# Autodesk Inventor assembly: assembly
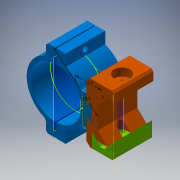
[picture p0: Inventor's stored thumbnail of the model, 180x180]
Saved by Autodesk Inventor 2019 (Build 230136000, 136)
## iProperties
Created: 2021-10-21
Part Number: assembly
Material: Genérico
Document SubType Name: Assembly
Designer: Juan M. Casillas
Author: Juan M. Casillas
## Documents named in this file (4)
- K:\3DPrinting\3DModels\RIS\assembly.iam
- K:\3DPrinting\3DModels\RIS\bolt_part.ipt
- K:\3DPrinting\3DModels\RIS\nut_part.ipt
- K:\3DPrinting\3DModels\RIS\flashlight_support.ipt
## Components (3 placed, 3 different names)
1. bolt_part:1 — Rigid:1, Rigid:2
2. nut_part:1 — Rigid:1
3. flashlight_support:1 — Rigid:2
## Relationships (2: WeldJoint 2)
- Rigid:1 [WeldJoint]: bolt_part:1 ↔ nut_part:1
- Rigid:2 [WeldJoint]: bolt_part:1 ↔ flashlight_support:1
